# Autodesk Inventor assembly: BrakeLight
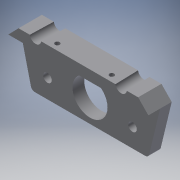
[picture p0: Inventor's stored thumbnail of the model, 180x180]
Saved by Autodesk Inventor 2019 (Build 230136000, 136)
## iProperties
Created: 2019-08-14
Part Number: BrakeLight
Document SubType Name: Assembly
Designer: steve
Author: steve
## Documents named in this file (3)
- C:\Users\steve\Documents\GitHub\Motorcycle\CAD Files\BrakeLight.iam
- C:\Users\steve\Documents\GitHub\Motorcycle\CAD Files\Brake_Light_Base_Plate.ipt
- C:\Users\steve\Documents\GitHub\Motorcycle\CAD Files\Bar_Mount_Bottom.ipt
## Components (2 placed, 2 different names)
1. Brake_Light_Base_Plate:1 — Rigid:1
2. Bar_Mount_Bottom:1 — Rigid:1
## Relationships (1: WeldJoint 1)
- Rigid:1 [WeldJoint]: Brake_Light_Base_Plate:1 ↔ Bar_Mount_Bottom:1
